# Autodesk Inventor assembly: 6P Sprocket
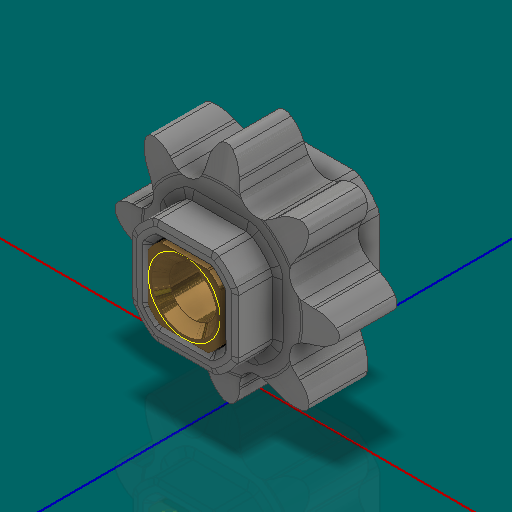
[picture p0: Inventor's stored thumbnail of the model, 512x512]
Saved by Autodesk Inventor 2025 (Build 290162000, 162)
## iProperties
Created: 2022-08-02
Part Number: 6P Sprocket
Document SubType Name: Assembly
Designer: ylu12
Author: ylu12
## Documents named in this file (4)
- C:\Users\avere\vex_robotics_high_stakes\hardware\cad\VEX-CAD-Inventor\Motion\Sprockets\6P Sprocket\6P 8T Sprocket, Circle.iam
- C:\Users\avere\vex_robotics_high_stakes\hardware\cad\VEX-CAD-Inventor\Motion\HS Shaft Adapter Circle.ipt
- C:\Users\avere\vex_robotics_high_stakes\hardware\cad\VEX-CAD-Inventor\Motion\Sprockets\Reference Files\6P 8T Sprocket.ipt
- C:\Users\avere\vex_robotics_high_stakes\hardware\cad\VEX-CAD-Inventor\Motion\Sprockets\6P Sprocket.iam
## Components (2 placed, 2 different names)
1. Circle — Flush:1, Mate:1, Mate:3
2. 8T — Mate:5, Mate:6, Flush:3
## Relationships (6: Mate 4, Flush 2)
- Flush:1 (6.35 mm): Circle
- Mate:1: Circle
- Mate:3: Circle
- Mate:5: 8T
- Mate:6: 8T
- Flush:3: 8T
